# Autodesk Inventor assembly: ensamble
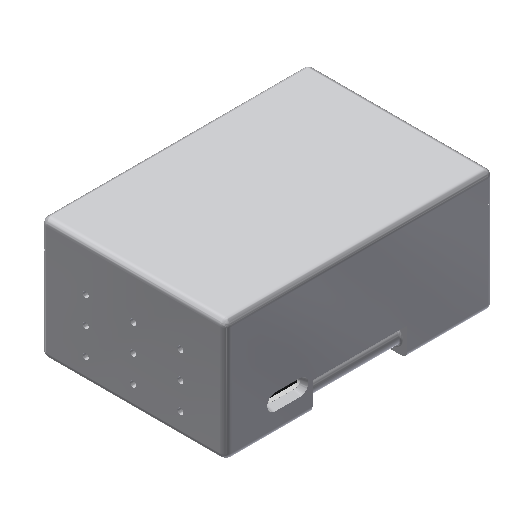
[picture p0: Inventor's stored thumbnail of the model, 512x512]
Saved by Autodesk Inventor 2025.2 (Build 292293000, 293)
## iProperties
Created: 2025-10-17
Part Number: ensamble
Material: Generic
Document SubType Name: Assembly
Designer: Ricardo
Author: Ricardo
## Documents named in this file (11)
- C:\Users\Ricardo\Documents\Inventor\TFC\ensamble.iam
- C:\Users\Ricardo\Documents\Inventor\TFC\Componentes\d-sun-dc-dc-step-down-voltage-regulator-simple-version-1.snapshot.4\PCB COMPLETA.iam
- C:\Users\Ricardo\Documents\Inventor\TFC\Base.ipt
- C:\Users\Ricardo\Documents\Inventor\TFC\Componentes\motor.ipt
- C:\Users\Ricardo\Documents\Inventor\TFC\Componentes\esp32_devkitv1-1.snapshot.7\ESP32_DevKitV1\ESP32_DevKitV1_en.ipt
- C:\Users\Ricardo\Documents\Inventor\TFC\superior.ipt
- C:\Users\Ricardo\Documents\Inventor\TFC\Componentes\523450-li-iron-battery-1000mah-3-7wh-dc4-2v-1.snapshot.13\523450 Li-iron Battery 1000mAh 3.7Wh DC4.2V\523450 Li-iron Battery 1000mAh 3.7Wh DC4.2V\Bateria.iam
- C:\Users\Ricardo\Documents\Inventor\TFC\Inserto Roscado.ipt
- C:\Users\Ricardo\Documents\Inventor\Content Center Files\R2025\en-US\ISO 7045(1)\DIN EN ISO 7045 - M2 x 6 - 4.8 - H.ipt
- C:\Users\Ricardo\Documents\Inventor\TFC\Componentes\push-switch-8x8-6pin-with-lock-1.snapshot.1\LatchSwitch_7x7\LatchSwitch_7x7\LatchSwitch_7x7_ens.ipt
- C:\Users\Ricardo\Documents\Inventor\TFC\Componentes\max30102-mh_et_live-board-1.snapshot.1\MAX30102_MH_ET_LIVE_BOARD_v8_ensamble.iam
## Components (16 placed, 10 different names)
1. PCB COMPLETA:1 [sub-assembly] — Mate:15, Mate:16, Mate:17, Mate:32, Mate:33, Mate:34, Insert:6, Insert:7, Insert:8, Insert:9
2. Base:1 — Mate:3, Flush:1, Flush:2, Mate:18, Insert:5, Mate:19, Mate:20, Mate:32, Mate:33, Mate:34, Mate:35, Flush:4, Mate:36, Flush:5, Mate:37, Flush:6, Flush:7, Mate:38, Flush:8, Mate:40, Mate:41, Flush:9, Mate:42, Flush:10, Mate:46, Mate:47
3. motor:1 — Mate:3, Insert:5
4. ESP32_DevKitV1_en:1 — Mate:15, Mate:16, Mate:17
5. superior:1 — Flush:1, Flush:2, Mate:18, Flush:8, Mate:42, Mate:43, Mate:44, Mate:45
6. Inserto Roscado:1 — Mate:35, Flush:4
7. Inserto Roscado:2 — Mate:36, Flush:5
8. Inserto Roscado:3 — Mate:37, Flush:6
9. Inserto Roscado:4 — Flush:7, Mate:38
10. DIN EN ISO 7045 H M2 x 6 - 4.8 - H:1 — Insert:6
11. DIN EN ISO 7045 H M2 x 6 - 4.8 - H:2 — Insert:7
12. DIN EN ISO 7045 H M2 x 6 - 4.8 - H:3 — Insert:8
13. DIN EN ISO 7045 H M2 x 6 - 4.8 - H:4 — Insert:9
14. LatchSwitch_7x7_ens:1 — Mate:40, Mate:41, Flush:9
15. Bateria:2 [sub-assembly] — Mate:43, Mate:44, Mate:45
16. MAX30102_MH_ET_LIVE_BOARD_v8_ensamble:1 [sub-assembly] — Flush:10, Mate:46, Mate:47
## Relationships (36: Mate 22, Flush 9, Insert 5)
- Mate:3: Base:1 ↔ motor:1
- Flush:1: Base:1 ↔ superior:1
- Flush:2: Base:1 ↔ superior:1
- Mate:15: PCB COMPLETA:1 ↔ ESP32_DevKitV1_en:1
- Mate:16: PCB COMPLETA:1 ↔ ESP32_DevKitV1_en:1
- Mate:17: PCB COMPLETA:1 ↔ ESP32_DevKitV1_en:1
- Mate:18: Base:1 ↔ superior:1
- Insert:5: Base:1 ↔ motor:1
- Mate:19: Base:1
- Mate:20: Base:1
- Mate:32: PCB COMPLETA:1 ↔ Base:1
- Mate:33 (0.5 mm): PCB COMPLETA:1 ↔ Base:1
- Mate:34 (1 mm): PCB COMPLETA:1 ↔ Base:1
- Mate:35: Base:1 ↔ Inserto Roscado:1
- Flush:4: Base:1 ↔ Inserto Roscado:1
- Mate:36: Base:1 ↔ Inserto Roscado:2
- Flush:5: Base:1 ↔ Inserto Roscado:2
- Mate:37: Base:1 ↔ Inserto Roscado:3
- Flush:6: Base:1 ↔ Inserto Roscado:3
- Flush:7: Base:1 ↔ Inserto Roscado:4
- Mate:38: Base:1 ↔ Inserto Roscado:4
- Insert:6: PCB COMPLETA:1 ↔ DIN EN ISO 7045 H M2 x 6 - 4.8 - H:1
- Insert:7: PCB COMPLETA:1 ↔ DIN EN ISO 7045 H M2 x 6 - 4.8 - H:2
- Insert:8: PCB COMPLETA:1 ↔ DIN EN ISO 7045 H M2 x 6 - 4.8 - H:3
- Insert:9: PCB COMPLETA:1 ↔ DIN EN ISO 7045 H M2 x 6 - 4.8 - H:4
- Flush:8: Base:1 ↔ superior:1
- Mate:40: Base:1 ↔ LatchSwitch_7x7_ens:1
- Mate:41: Base:1 ↔ LatchSwitch_7x7_ens:1
- Flush:9: Base:1 ↔ LatchSwitch_7x7_ens:1
- Mate:42: Base:1 ↔ superior:1
- Mate:43: superior:1 ↔ Bateria:2
- Mate:44: superior:1 ↔ Bateria:2
- Mate:45: superior:1 ↔ Bateria:2
- Flush:10: Base:1 ↔ MAX30102_MH_ET_LIVE_BOARD_v8_ensamble:1
- Mate:46: Base:1 ↔ MAX30102_MH_ET_LIVE_BOARD_v8_ensamble:1
- Mate:47: Base:1 ↔ MAX30102_MH_ET_LIVE_BOARD_v8_ensamble:1
